# Autodesk Inventor assembly: tubing_alignment_assembly
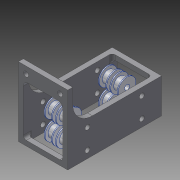
[picture p0: Inventor's stored thumbnail of the model, 180x180]
Saved by Autodesk Inventor 2015 (Build 190159000, 159)
## iProperties
Created: 2017-04-14
Part Number: tubing_alignment_assembly
Document SubType Name: Assembly
Designer: Guy
Author: Guy
## Documents named in this file (3)
- C:\Users\Guy\Documents\Fourth Year\Capstone\git\Capstone-Project\doc\CAD\LowLevel_Rev3\tubing_alignment_assembly.iam
- C:\Users\Guy\Documents\Fourth Year\Capstone\git\Capstone-Project\doc\CAD\LowLevel_Rev3\tubing_alignment_arm[2].ipt
- C:\Users\Guy\Documents\Fourth Year\Capstone\git\Capstone-Project\doc\CAD\LowLevel_Rev3\XY_Wheel-SquareBar-Rev3.ipt
## Components (9 placed, 2 different names)
1. tubing_alignment_arm[2]:1 — Mate:1, Mate:2, Mate:3, Mate:4, Mate:5, Mate:6, Mate:7, Mate:8, Mate:9, Mate:10, Mate:11, Mate:12, Mate:13, Mate:14, Mate:15, Mate:16
2. XY_Wheel-SquareBar-Rev3:1 — Mate:1, Mate:9
3. XY_Wheel-SquareBar-Rev3:2 — Mate:2, Mate:10
4. XY_Wheel-SquareBar-Rev3:3 — Mate:3, Mate:15
5. XY_Wheel-SquareBar-Rev3:4 — Mate:4, Mate:16
6. XY_Wheel-SquareBar-Rev3:5 — Mate:7, Mate:11
7. XY_Wheel-SquareBar-Rev3:6 — Mate:8, Mate:12
8. XY_Wheel-SquareBar-Rev3:7 — Mate:5, Mate:14
9. XY_Wheel-SquareBar-Rev3:8 — Mate:6, Mate:13
## Relationships (16: Mate 16)
- Mate:1: tubing_alignment_arm[2]:1 ↔ XY_Wheel-SquareBar-Rev3:1
- Mate:2: tubing_alignment_arm[2]:1 ↔ XY_Wheel-SquareBar-Rev3:2
- Mate:3: tubing_alignment_arm[2]:1 ↔ XY_Wheel-SquareBar-Rev3:3
- Mate:4: tubing_alignment_arm[2]:1 ↔ XY_Wheel-SquareBar-Rev3:4
- Mate:5: tubing_alignment_arm[2]:1 ↔ XY_Wheel-SquareBar-Rev3:7
- Mate:6: tubing_alignment_arm[2]:1 ↔ XY_Wheel-SquareBar-Rev3:8
- Mate:7: tubing_alignment_arm[2]:1 ↔ XY_Wheel-SquareBar-Rev3:5
- Mate:8: tubing_alignment_arm[2]:1 ↔ XY_Wheel-SquareBar-Rev3:6
- Mate:9 (10 mm): tubing_alignment_arm[2]:1 ↔ XY_Wheel-SquareBar-Rev3:1
- Mate:10 (10 mm): tubing_alignment_arm[2]:1 ↔ XY_Wheel-SquareBar-Rev3:2
- Mate:11 (10 mm): tubing_alignment_arm[2]:1 ↔ XY_Wheel-SquareBar-Rev3:5
- Mate:12 (10 mm): tubing_alignment_arm[2]:1 ↔ XY_Wheel-SquareBar-Rev3:6
- Mate:13 (10 mm): tubing_alignment_arm[2]:1 ↔ XY_Wheel-SquareBar-Rev3:8
- Mate:14 (10 mm): tubing_alignment_arm[2]:1 ↔ XY_Wheel-SquareBar-Rev3:7
- Mate:15 (10 mm): tubing_alignment_arm[2]:1 ↔ XY_Wheel-SquareBar-Rev3:3
- Mate:16 (10 mm): tubing_alignment_arm[2]:1 ↔ XY_Wheel-SquareBar-Rev3:4
